# Autodesk Inventor assembly: Редуктор
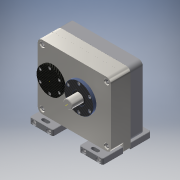
[picture p0: Inventor's stored thumbnail of the model, 180x180]
Saved by Autodesk Inventor 2016 (Build 200138000, 138)
## iProperties
Created: 2021-04-28
Part Number: Редуктор
Material: Типовые
Document SubType Name: Assembly
Designer: Лол
Author: Лол
## Documents named in this file (30)
- C:\Users\Лол\Documents\Inventor\course_work\Редуктор.iam
- C:\Users\Лол\Documents\Inventor\course_work\Корпус часть без резьбы.ipt
- C:\Users\Лол\Documents\Inventor\course_work\Подшипник\Подшипник-01.ipt
- C:\Users\Лол\Documents\Inventor\course_work\Подшипник.ipt
- C:\Users\Лол\Documents\Inventor\course_work\Подшипник\Подшипник-02.ipt
- C:\Users\Лол\Documents\Inventor\course_work\Быстроходный вал.ipt
- C:\Users\Лол\Documents\Inventor\course_work\Тихоходный вал.ipt
- C:\Users\Лол\Documents\Inventor\course_work\Кольцо A30 ГОСТ 13942-86.ipt
- C:\Users\Лол\Documents\Inventor\course_work\Кольцо A35 ГОСТ 13942-86.ipt
- C:\Users\Лол\Documents\Inventor\course_work\Тихоходное колесо.ipt
- C:\Users\Лол\Documents\Inventor\course_work\Корпус центральная часть.ipt
- C:\Users\Лол\Documents\Inventor\course_work\Корпус часть с резьбой.ipt
- C:\Users\Лол\Documents\Inventor\course_work\Гайка M30x1.5 6H ГОСТ 6393-73.ipt
- C:\Users\Лол\Documents\Inventor\course_work\Гайка M33x1.5 6H ГОСТ 6393-73.ipt
- C:\Users\Лол\Documents\Inventor\course_work\ISO 2340 - A - 6 x 40ISO.ipt
- C:\Users\Лол\Documents\Inventor\course_work\AS 1420 - 1973 - M10 x 75.ipt
- C:\Users\Лол\Documents\Inventor\course_work\Крышка маленькая_62.ipt
- C:\Users\Лол\Documents\Inventor\course_work\КОЛЬЦО 062-066-25 гост 9833.ipt
- C:\Users\Лол\Documents\Inventor\course_work\Манжет 1-30x72x10 ГОСТ 8752-79.ipt
- C:\Users\Лол\Documents\Inventor\course_work\Манжет 1-28x62x10 ГОСТ 8752-79.ipt
- C:\Users\Лол\Documents\Inventor\course_work\Крышка большая_72.ipt
- C:\Users\Лол\Documents\Inventor\course_work\КОЛЬЦО 072-066-25 гост 9833.ipt
- C:\Users\Лол\Documents\Inventor\course_work\AS 1420 - 1973 - M6 x 12.ipt
- C:\Users\Лол\Documents\Inventor\course_work\ОПОРА_01.ipt
- C:\Users\Лол\Documents\Inventor\course_work\ОПОРА_02.ipt
- C:\Users\Лол\Documents\Inventor\course_work\Крышка маленькая_под манж_01.ipt
- C:\Users\Лол\Documents\Inventor\course_work\Крышка большая_ПОД МАНЖЕТУ.ipt
- C:\Users\Лол\Documents\Inventor\course_work\Манжет 1-28x40x7 ГОСТ 8752-79.ipt
- C:\Users\Лол\Documents\Inventor\course_work\Манжет 1-30x42x7 ГОСТ 8752-79.ipt
- C:\Users\Лол\Documents\Inventor\course_work\AS 1420 - 1973 - M10 x 80.ipt
## Components (68 placed, 28 different names)
1. Корпус часть без резьбы:1 — Заподлицо:1, Заподлицо:2, Заподлицо:3, Совмещение:1, Совмещение:2, Совмещение:3, Совмещение:4, Совмещение:14, Совмещение:27, Совмещение:28, Совмещение:33, Совмещение:34, Совмещение:35, Совмещение:36, Совмещение:37, Совмещение:38, Совмещение:39, Совмещение:40, Совмещение:43, Совмещение:44, Совмещение:46, Заподлицо:4, Совмещение:61, Совмещение:62, Совмещение:82, Совмещение:83, Совмещение:84
2. Подшипник-01:1 — Совмещение:18, Совмещение:19, Совмещение:22, Совмещение:24
3. Подшипник-01:2 — Совмещение:1, Совмещение:2, Совмещение:5, Совмещение:13
4. Подшипник-02:3 — Совмещение:3, Совмещение:4, Совмещение:6, Совмещение:26
5. Подшипник-02:4 — Совмещение:16, Совмещение:17, Совмещение:, Совмещение:88
6. Быстроходный вал:1 — Совмещение:5, Совмещение:7, Совмещение:8, Совмещение:22, Совмещение:23, Совмещение:85, Совмещение:109
7. Тихоходный вал:1 — Совмещение:6, Совмещение:9, Совмещение:12, Совмещение:25, Совмещение:48, Совмещение:87, Совмещение:88, Совмещение:112
8. Кольцо A30 ГОСТ 13942-86:1 — Совмещение:7, Совмещение:8, Совмещение:13
9. Кольцо A35 ГОСТ 13942-86:1 — Совмещение:9, Совмещение:, Совмещение:48
10. Тихоходное колесо:2 — Совмещение:12, Совмещение:87
11. Корпус центральная часть:1 — Совмещение:14, Совмещение:15, Совмещение:29, Совмещение:30, Совмещение:31, Совмещение:32, Совмещение:67, Совмещение:68, Совмещение:69, Совмещение:70, Совмещение:71, Совмещение:72, Совмещение:73, Совмещение:74, Совмещение:75, Совмещение:76, Совмещение:77, Совмещение:78, Совмещение:91, Заподлицо:8, Совмещение:92, Совмещение:93, Совмещение:94, Совмещение:95, Совмещение:96, Заподлицо:9
12. Корпус часть с резьбой:1 — Совмещение:15, Совмещение:16, Совмещение:17, Совмещение:18, Совмещение:19, Совмещение:47, Заподлицо:5, Совмещение:49, Совмещение:56, Совмещение:57, Совмещение:65, Совмещение:79, Совмещение:80, Совмещение:81
13. Гайка M30x1.5 6H ГОСТ 6393-73:1 — Совмещение:23, Совмещение:24
14. Гайка M33x1.5 6H ГОСТ 6393-73:1 — Совмещение:25, Совмещение:26
15. ISO 2340 - A - 6 x 40ISO:1 — Совмещение:27, Совмещение:29, Совмещение:31
16. ISO 2340 - A - 6 x 40ISO:2 — Совмещение:28, Совмещение:30, Совмещение:32
17. AS 1420 - 1973 - M10 x 75:1 — Совмещение:33, Совмещение:34
18. AS 1420 - 1973 - M10 x 75:2 — Совмещение:35, Совмещение:36
19. AS 1420 - 1973 - M10 x 75:3 — Совмещение:37, Совмещение:38
20. AS 1420 - 1973 - M10 x 75:4 — Совмещение:39, Совмещение:40
21. Крышка маленькая_62:1 — Совмещение:41, Совмещение:42, Совмещение:43, Совмещение:44, Совмещение:61, Совмещение:63, Совмещение:64
22. КОЛЬЦО 062-066-25 гост 9833:1 — Совмещение:41, Совмещение:42
23. Манжет 1-30x72x10 ГОСТ 8752-79:2 — Совмещение:46, Заподлицо:4
24. Манжет 1-28x62x10 ГОСТ 8752-79:2 — Совмещение:47, Заподлицо:5
25. Крышка большая_72:2 — Совмещение:49, Совмещение:50, Совмещение:51, Совмещение:56, Совмещение:57, Совмещение:60, Совмещение:66
26. КОЛЬЦО 072-066-25 гост 9833:1 — Совмещение:50, Совмещение:51
27. ОПОРА_01:1 — Совмещение:67, Совмещение:68, Совмещение:69, Совмещение:98, Совмещение:99, Совмещение:100, Совмещение:102
28. ОПОРА_01:2 — Совмещение:70, Совмещение:71, Совмещение:72, Совмещение:89, Совмещение:90, Совмещение:97, Совмещение:101
29. ОПОРА_02:1 — Совмещение:76, Совмещение:77, Совмещение:78
30. ОПОРА_02:2 — Совмещение:73, Совмещение:74, Совмещение:75
31. Крышка маленькая_под манж_01:1 — Совмещение:79, Совмещение:80, Совмещение:81, Заподлицо:6, Совмещение:105, Совмещение:106, Совмещение:107, Совмещение:108
32. Крышка большая_ПОД МАНЖЕТУ:1 — Совмещение:82, Совмещение:83, Совмещение:84, Заподлицо:7, Совмещение:86, Совмещение:103, Совмещение:104, Совмещение:110, Совмещение:111
33. Манжет 1-28x40x7 ГОСТ 8752-79:2 — Совмещение:85, Заподлицо:6
34. Манжет 1-30x42x7 ГОСТ 8752-79:1 — Заподлицо:7, Совмещение:86
35. AS 1420 - 1973 - M10 x 80:1 — Совмещение:89, Совмещение:90
36. ISO 2340 - A - 6 x 40ISO:3 — Совмещение:91, Заподлицо:8
37. ISO 2340 - A - 6 x 40ISO:4 — Совмещение:92, Совмещение:95
38. ISO 2340 - A - 6 x 40ISO:5 — Совмещение:93, Совмещение:96
39. ISO 2340 - A - 6 x 40ISO:6 — Совмещение:94, Заподлицо:9
40. AS 1420 - 1973 - M10 x 80:2 — Совмещение:97, Совмещение:101
41. AS 1420 - 1973 - M10 x 80:3 — Совмещение:98, Совмещение:100
42. AS 1420 - 1973 - M10 x 80:4 — Совмещение:99, Совмещение:102
43. КОЛЬЦО 072-066-25 гост 9833:2 — Совмещение:103, Совмещение:104
44. КОЛЬЦО 062-066-25 гост 9833:2 — Совмещение:105, Совмещение:106
45. AS 1420 - 1973 - M6 x 12:1 — Совмещение:62, Совмещение:63
46. AS 1420 - 1973 - M6 x 12:2
47. AS 1420 - 1973 - M6 x 12:3
48. AS 1420 - 1973 - M6 x 12:4
49. AS 1420 - 1973 - M6 x 12:5
50. AS 1420 - 1973 - M6 x 12:6
51. AS 1420 - 1973 - M6 x 12:8 — Совмещение:65, Совмещение:66
52. AS 1420 - 1973 - M6 x 12:9
53. AS 1420 - 1973 - M6 x 12:10
54. AS 1420 - 1973 - M6 x 12:11
55. AS 1420 - 1973 - M6 x 12:12
56. AS 1420 - 1973 - M6 x 12:13
57. AS 1420 - 1973 - M6 x 12:15 — Совмещение:107, Совмещение:108
58. AS 1420 - 1973 - M6 x 12:16
59. AS 1420 - 1973 - M6 x 12:17
60. AS 1420 - 1973 - M6 x 12:18
61. AS 1420 - 1973 - M6 x 12:19
62. AS 1420 - 1973 - M6 x 12:20
63. AS 1420 - 1973 - M6 x 12:14 — Совмещение:110, Совмещение:111
64. AS 1420 - 1973 - M6 x 12:21
65. AS 1420 - 1973 - M6 x 12:22
66. AS 1420 - 1973 - M6 x 12:23
67. AS 1420 - 1973 - M6 x 12:24
68. AS 1420 - 1973 - M6 x 12:25
## Component patterns: (6 elements, first: AS 1420 - 1973 - M6 x 12:1), (6 elements, first: AS 1420 - 1973 - M6 x 12:8), (6 elements, first: AS 1420 - 1973 - M6 x 12:15), (6 elements, first: AS 1420 - 1973 - M6 x 12:14)
## Relationships (111: Mate 102, Flush 9)
- Заподлицо:1 [Flush]: Корпус часть без резьбы:1
- Заподлицо:2 [Flush] (-37.142 mm): Корпус часть без резьбы:1
- Заподлицо:3 [Flush] (-27.571 mm): Корпус часть без резьбы:1
- Совмещение:1 [Mate]: Корпус часть без резьбы:1 ↔ Подшипник-01:2
- Совмещение:2 [Mate]: Корпус часть без резьбы:1 ↔ Подшипник-01:2
- Совмещение:3 [Mate]: Корпус часть без резьбы:1 ↔ Подшипник-02:3
- Совмещение:4 [Mate]: Корпус часть без резьбы:1 ↔ Подшипник-02:3
- Совмещение:5 [Mate]: Подшипник-01:2 ↔ Быстроходный вал:1
- Совмещение:6 [Mate]: Подшипник-02:3 ↔ Тихоходный вал:1
- Совмещение:7 [Mate]: Быстроходный вал:1 ↔ Кольцо A30 ГОСТ 13942-86:1
- Совмещение:8 [Mate]: Быстроходный вал:1 ↔ Кольцо A30 ГОСТ 13942-86:1
- Совмещение:9 [Mate]: Тихоходный вал:1 ↔ Кольцо A35 ГОСТ 13942-86:1
- Совмещение:12 [Mate]: Тихоходный вал:1 ↔ Тихоходное колесо:2
- Совмещение:13 [Mate]: Подшипник-01:2 ↔ Кольцо A30 ГОСТ 13942-86:1
- Совмещение:14 [Mate]: Корпус часть без резьбы:1 ↔ Корпус центральная часть:1
- Совмещение:15 [Mate]: Корпус центральная часть:1 ↔ Корпус часть с резьбой:1
- Совмещение:16 [Mate]: Подшипник-02:4 ↔ Корпус часть с резьбой:1
- Совмещение:17 [Mate]: Подшипник-02:4 ↔ Корпус часть с резьбой:1
- Совмещение:18 [Mate]: Подшипник-01:1 ↔ Корпус часть с резьбой:1
- Совмещение:19 [Mate]: Подшипник-01:1 ↔ Корпус часть с резьбой:1
- Совмещение: [Mate]: Подшипник-02:4 ↔ Кольцо A35 ГОСТ 13942-86:1
- Совмещение:22 [Mate]: Подшипник-01:1 ↔ Быстроходный вал:1
- Совмещение:23 [Mate]: Быстроходный вал:1 ↔ Гайка M30x1.5 6H ГОСТ 6393-73:1
- Совмещение:24 [Mate]: Подшипник-01:1 ↔ Гайка M30x1.5 6H ГОСТ 6393-73:1
- Совмещение:25 [Mate]: Тихоходный вал:1 ↔ Гайка M33x1.5 6H ГОСТ 6393-73:1
- Совмещение:26 [Mate]: Подшипник-02:3 ↔ Гайка M33x1.5 6H ГОСТ 6393-73:1
- Совмещение:27 [Mate]: Корпус часть без резьбы:1 ↔ ISO 2340 - A - 6 x 40ISO:1
- Совмещение:28 [Mate]: Корпус часть без резьбы:1 ↔ ISO 2340 - A - 6 x 40ISO:2
- Совмещение:29 [Mate]: Корпус центральная часть:1 ↔ ISO 2340 - A - 6 x 40ISO:1
- Совмещение:30 [Mate]: Корпус центральная часть:1 ↔ ISO 2340 - A - 6 x 40ISO:2
- Совмещение:31 [Mate] (7.5 mm): Корпус центральная часть:1 ↔ ISO 2340 - A - 6 x 40ISO:1
- Совмещение:32 [Mate] (7.5 mm): Корпус центральная часть:1 ↔ ISO 2340 - A - 6 x 40ISO:2
- Совмещение:33 [Mate]: Корпус часть без резьбы:1 ↔ AS 1420 - 1973 - M10 x 75:1
- Совмещение:34 [Mate]: Корпус часть без резьбы:1 ↔ AS 1420 - 1973 - M10 x 75:1
- Совмещение:35 [Mate]: Корпус часть без резьбы:1 ↔ AS 1420 - 1973 - M10 x 75:2
- Совмещение:36 [Mate]: Корпус часть без резьбы:1 ↔ AS 1420 - 1973 - M10 x 75:2
- Совмещение:37 [Mate]: Корпус часть без резьбы:1 ↔ AS 1420 - 1973 - M10 x 75:3
- Совмещение:38 [Mate]: Корпус часть без резьбы:1 ↔ AS 1420 - 1973 - M10 x 75:3
- Совмещение:39 [Mate]: Корпус часть без резьбы:1 ↔ AS 1420 - 1973 - M10 x 75:4
- Совмещение:40 [Mate]: Корпус часть без резьбы:1 ↔ AS 1420 - 1973 - M10 x 75:4
- Совмещение:41 [Mate]: Крышка маленькая_62:1 ↔ КОЛЬЦО 062-066-25 гост 9833:1
- Совмещение:42 [Mate] (1.25 mm): Крышка маленькая_62:1 ↔ КОЛЬЦО 062-066-25 гост 9833:1
- Совмещение:43 [Mate]: Корпус часть без резьбы:1 ↔ Крышка маленькая_62:1
- Совмещение:44 [Mate]: Корпус часть без резьбы:1 ↔ Крышка маленькая_62:1
- Совмещение:46 [Mate]: Корпус часть без резьбы:1 ↔ Манжет 1-30x72x10 ГОСТ 8752-79:2
- Заподлицо:4 [Flush]: Корпус часть без резьбы:1 ↔ Манжет 1-30x72x10 ГОСТ 8752-79:2
- Совмещение:47 [Mate]: Корпус часть с резьбой:1 ↔ Манжет 1-28x62x10 ГОСТ 8752-79:2
- Заподлицо:5 [Flush]: Корпус часть с резьбой:1 ↔ Манжет 1-28x62x10 ГОСТ 8752-79:2
- Совмещение:48 [Mate]: Тихоходный вал:1 ↔ Кольцо A35 ГОСТ 13942-86:1
- Совмещение:49 [Mate]: Корпус часть с резьбой:1 ↔ Крышка большая_72:2
- Совмещение:50 [Mate]: Крышка большая_72:2 ↔ КОЛЬЦО 072-066-25 гост 9833:1
- Совмещение:51 [Mate] (1.25 mm): Крышка большая_72:2 ↔ КОЛЬЦО 072-066-25 гост 9833:1
- Совмещение:56 [Mate]: Корпус часть с резьбой:1 ↔ Крышка большая_72:2
- Совмещение:57 [Mate]: Корпус часть с резьбой:1 ↔ Крышка большая_72:2
- Совмещение:60 [Mate]: Крышка большая_72:2
- Совмещение:61 [Mate]: Корпус часть без резьбы:1 ↔ Крышка маленькая_62:1
- Совмещение:62 [Mate]: Корпус часть без резьбы:1 ↔ AS 1420 - 1973 - M6 x 12:1
- Совмещение:63 [Mate]: Крышка маленькая_62:1 ↔ AS 1420 - 1973 - M6 x 12:1
- Совмещение:64 [Mate]: Крышка маленькая_62:1
- Совмещение:65 [Mate]: Корпус часть с резьбой:1 ↔ AS 1420 - 1973 - M6 x 12:8
- Совмещение:66 [Mate]: Крышка большая_72:2 ↔ AS 1420 - 1973 - M6 x 12:8
- Совмещение:67 [Mate]: Корпус центральная часть:1 ↔ ОПОРА_01:1
- Совмещение:68 [Mate]: Корпус центральная часть:1 ↔ ОПОРА_01:1
- Совмещение:69 [Mate]: Корпус центральная часть:1 ↔ ОПОРА_01:1
- Совмещение:70 [Mate]: Корпус центральная часть:1 ↔ ОПОРА_01:2
- Совмещение:71 [Mate]: Корпус центральная часть:1 ↔ ОПОРА_01:2
- Совмещение:72 [Mate]: Корпус центральная часть:1 ↔ ОПОРА_01:2
- Совмещение:73 [Mate]: Корпус центральная часть:1 ↔ ОПОРА_02:2
- Совмещение:74 [Mate]: Корпус центральная часть:1 ↔ ОПОРА_02:2
- Совмещение:75 [Mate]: Корпус центральная часть:1 ↔ ОПОРА_02:2
- Совмещение:76 [Mate]: Корпус центральная часть:1 ↔ ОПОРА_02:1
- Совмещение:77 [Mate]: Корпус центральная часть:1 ↔ ОПОРА_02:1
- Совмещение:78 [Mate]: Корпус центральная часть:1 ↔ ОПОРА_02:1
- Совмещение:79 [Mate]: Корпус часть с резьбой:1 ↔ Крышка маленькая_под манж_01:1
- Совмещение:80 [Mate]: Корпус часть с резьбой:1 ↔ Крышка маленькая_под манж_01:1
- Совмещение:81 [Mate]: Корпус часть с резьбой:1 ↔ Крышка маленькая_под манж_01:1
- Совмещение:82 [Mate]: Корпус часть без резьбы:1 ↔ Крышка большая_ПОД МАНЖЕТУ:1
- Совмещение:83 [Mate]: Корпус часть без резьбы:1 ↔ Крышка большая_ПОД МАНЖЕТУ:1
- Совмещение:84 [Mate]: Корпус часть без резьбы:1 ↔ Крышка большая_ПОД МАНЖЕТУ:1
- Совмещение:85 [Mate]: Быстроходный вал:1 ↔ Манжет 1-28x40x7 ГОСТ 8752-79:2
- Заподлицо:6 [Flush]: Крышка маленькая_под манж_01:1 ↔ Манжет 1-28x40x7 ГОСТ 8752-79:2
- Заподлицо:7 [Flush]: Крышка большая_ПОД МАНЖЕТУ:1 ↔ Манжет 1-30x42x7 ГОСТ 8752-79:1
- Совмещение:86 [Mate]: Крышка большая_ПОД МАНЖЕТУ:1 ↔ Манжет 1-30x42x7 ГОСТ 8752-79:1
- Совмещение:87 [Mate]: Тихоходный вал:1 ↔ Тихоходное колесо:2
- Совмещение:88 [Mate]: Подшипник-02:4 ↔ Тихоходный вал:1
- Совмещение:89 [Mate]: ОПОРА_01:2 ↔ AS 1420 - 1973 - M10 x 80:1
- Совмещение:90 [Mate]: ОПОРА_01:2 ↔ AS 1420 - 1973 - M10 x 80:1
- Совмещение:91 [Mate]: Корпус центральная часть:1 ↔ ISO 2340 - A - 6 x 40ISO:3
- Заподлицо:8 [Flush] (7.5 mm): Корпус центральная часть:1 ↔ ISO 2340 - A - 6 x 40ISO:3
- Совмещение:92 [Mate]: Корпус центральная часть:1 ↔ ISO 2340 - A - 6 x 40ISO:4
- Совмещение:93 [Mate]: Корпус центральная часть:1 ↔ ISO 2340 - A - 6 x 40ISO:5
- Совмещение:94 [Mate]: Корпус центральная часть:1 ↔ ISO 2340 - A - 6 x 40ISO:6
- Совмещение:95 [Mate] (7.5 mm): Корпус центральная часть:1 ↔ ISO 2340 - A - 6 x 40ISO:4
- Совмещение:96 [Mate] (7.5 mm): Корпус центральная часть:1 ↔ ISO 2340 - A - 6 x 40ISO:5
- Заподлицо:9 [Flush] (7.5 mm): Корпус центральная часть:1 ↔ ISO 2340 - A - 6 x 40ISO:6
- Совмещение:97 [Mate]: ОПОРА_01:2 ↔ AS 1420 - 1973 - M10 x 80:2
- Совмещение:98 [Mate]: ОПОРА_01:1 ↔ AS 1420 - 1973 - M10 x 80:3
- Совмещение:99 [Mate]: ОПОРА_01:1 ↔ AS 1420 - 1973 - M10 x 80:4
- Совмещение:100 [Mate]: ОПОРА_01:1 ↔ AS 1420 - 1973 - M10 x 80:3
- Совмещение:101 [Mate]: ОПОРА_01:2 ↔ AS 1420 - 1973 - M10 x 80:2
- Совмещение:102 [Mate]: ОПОРА_01:1 ↔ AS 1420 - 1973 - M10 x 80:4
- Совмещение:103 [Mate]: Крышка большая_ПОД МАНЖЕТУ:1 ↔ КОЛЬЦО 072-066-25 гост 9833:2
- Совмещение:104 [Mate] (1.25 mm): Крышка большая_ПОД МАНЖЕТУ:1 ↔ КОЛЬЦО 072-066-25 гост 9833:2
- Совмещение:105 [Mate]: Крышка маленькая_под манж_01:1 ↔ КОЛЬЦО 062-066-25 гост 9833:2
- Совмещение:106 [Mate] (1.25 mm): Крышка маленькая_под манж_01:1 ↔ КОЛЬЦО 062-066-25 гост 9833:2
- Совмещение:107 [Mate]: Крышка маленькая_под манж_01:1 ↔ AS 1420 - 1973 - M6 x 12:15
- Совмещение:108 [Mate]: Крышка маленькая_под манж_01:1 ↔ AS 1420 - 1973 - M6 x 12:15
- Совмещение:109 [Mate]: Быстроходный вал:1
- Совмещение:110 [Mate]: Крышка большая_ПОД МАНЖЕТУ:1 ↔ AS 1420 - 1973 - M6 x 12:14
- Совмещение:111 [Mate]: Крышка большая_ПОД МАНЖЕТУ:1 ↔ AS 1420 - 1973 - M6 x 12:14
- Совмещение:112 [Mate]: Тихоходный вал:1
